# Autodesk Inventor assembly: carriage
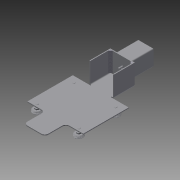
[picture p0: Inventor's stored thumbnail of the model, 180x180]
Saved by Autodesk Inventor 2013 (Build 170138000, 138)
## iProperties
Created: 2012-12-03
Part Number: carriage
Document SubType Name: Weldment
Designer: Istvan
Weld Material: Aluminum 6061, Welded
Author: Istvan
## Documents named in this file (5)
- D:\GitHub\Crown-Fire\CAD\Frame\y-carriage\carriage.iam
- D:\GitHub\Crown-Fire\CAD\Frame\y-carriage\backplate.ipt
- D:\GitHub\Crown-Fire\CAD\Hardware\Bearings\DualVee-size2.ipt
- D:\GitHub\Crown-Fire\CAD\Electronics\Motors\G723-280-4.ipt
- D:\GitHub\Crown-Fire\CAD\Frame\y-carriage\zMotorMount.ipt
## Components (7 placed, 4 different names)
1. backplate:1 — Mate:1, Mate:2, Mate:3, Mate:4, Mate:5, Flush:4, Flush:5
2. DualVee-size2:1 — Mate:3, Flush:1, Flush:2, Flush:3
3. DualVee-size2:2 — Mate:4, Flush:1
4. DualVee-size2:3 — Mate:2, Flush:3
5. DualVee-size2:4 — Mate:1, Flush:2
6. G723-280-4:1 — Mate:6, Mate:7
7. zMotorMount:1 — Mate:5, Flush:4, Flush:5, Mate:6, Mate:7
## Relationships (12: Mate 7, Flush 5)
- Mate:1: backplate:1 ↔ DualVee-size2:4
- Mate:2: backplate:1 ↔ DualVee-size2:3
- Mate:3: backplate:1 ↔ DualVee-size2:1
- Mate:4: backplate:1 ↔ DualVee-size2:2
- Flush:1: DualVee-size2:1 ↔ DualVee-size2:2
- Flush:2: DualVee-size2:1 ↔ DualVee-size2:4
- Flush:3: DualVee-size2:1 ↔ DualVee-size2:3
- Mate:5: backplate:1 ↔ zMotorMount:1
- Flush:4: backplate:1 ↔ zMotorMount:1
- Flush:5: backplate:1 ↔ zMotorMount:1
- Mate:6: G723-280-4:1 ↔ zMotorMount:1
- Mate:7 (5.08 mm): G723-280-4:1 ↔ zMotorMount:1
